# Autodesk Inventor assembly: mg996r leg top
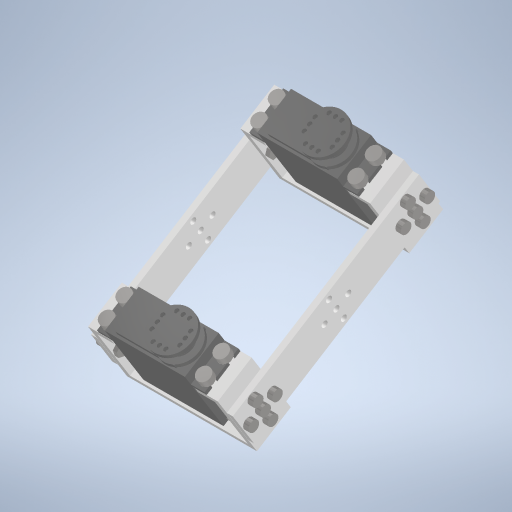
[picture p0: Inventor's stored thumbnail of the model, 512x512]
Saved by Autodesk Inventor 2023 (Build 270158000, 158)
## iProperties
Created: 2022-06-29
Part Number: mg996r leg top
Document SubType Name: Assembly
Designer: isamu
Author: isamu
## iProperties of the stored document Body008.ipt
Created: 2022-06-29
Part Number: Body008
Material: Generic
Document SubType Name: Modeling
Designer: isamu
Density: 1 g/cm^3
Appearance: Default
Author: isamu
## iProperties of the stored document servo frame part 4.iam
Created: 2022-07-03
Part Number: servo frame part 4
Description: FreeCAD Model
Document SubType Name: Assembly
Designer: isamu
Authority: Unknown
Sending System: FreeCAD
Preprocessor: Open CASCADE STEP processor 7.5
Title: Open CASCADE Shape Model
Author: Author
## Documents named in this file (7)
- **D:\personal_projects\robot\inventor\mg996r leg top.iam*LocalDocs*xAaaaafcaAaaaaaaaAaaaai2oXe*Body008.ipt
- **D:\personal_projects\robot\inventor\mg996r leg top.iam*LocalDocs*xAaaaajdaAaaaaaaaAaaaabubYc*servo frame part 4.iam
- D:\personal_projects\robot\inventor\mg996r leg top.iam
- D:\personal_projects\robot\exports\frames\m3x8.ipt
- D:\personal_projects\robot\exports\frames\m3 nuts.ipt
- D:\personal_projects\robot\inventor\base mg996r 3mm frame without axis.iam
- D:\personal_projects\robot\exports\frames\servo frame part 4.step
## Components (44 placed, 4 different names)
1. servo frame part 4:1 [sub-assembly] — Insert:26, Insert:27, Insert:28, Insert:29, Insert:30, Mate:1, Mate:7, Mate:8, Mate:9, Insert:41, Insert:42, Insert:43, Insert:44, Insert:45
2. servo frame part 4:2 [sub-assembly] — Insert:21, Insert:22, Insert:23, Insert:24, Insert:25, Mate:4, Insert:46, Insert:47, Insert:48, Insert:49, Insert:50
3. m3x8:1 — Insert:22, Mate:6
4. m3x8:2 — Insert:21, Mate:5
5. m3x8:3 — Insert:25
6. m3x8:4 — Insert:23
7. m3x8:5 — Insert:24
8. m3x8:6 — Insert:26, Mate:3
9. m3x8:7 — Insert:29
10. m3x8:8 — Insert:30
11. m3x8:9 — Insert:27, Mate:2
12. m3x8:10 — Insert:28
13. m3 nuts:1 — Insert:37
14. m3 nuts:2 — Insert:39
15. m3 nuts:3 — Insert:40
16. m3 nuts:4 — Insert:38
17. m3 nuts:5 — Insert:36
18. m3 nuts:6 — Insert:34
19. m3 nuts:7 — Insert:31
20. m3 nuts:8 — Insert:32
21. m3 nuts:9 — Insert:35
22. m3 nuts:10 — Insert:33
23. base mg996r 3mm frame without axis:1 [sub-assembly] — Mate:1, Mate:2, Mate:3, Mate:4, Mate:5, Mate:6, Insert:31, Insert:32, Insert:33, Insert:34, Insert:35, Insert:36, Insert:37, Insert:38, Insert:39, Insert:40
24. base mg996r 3mm frame without axis:2 [sub-assembly] — Mate:7, Mate:8, Mate:9, Insert:51, Insert:52, Insert:53, Insert:54, Insert:55, Insert:56, Insert:57, Insert:58, Insert:59, Insert:60
25. m3x8:11 — Insert:43
26. m3x8:12 — Insert:42
27. m3x8:13 — Insert:41
28. m3x8:14 — Insert:45
29. m3x8:15 — Insert:44
30. m3x8:16 — Insert:50
31. m3x8:17 — Insert:46
32. m3x8:18 — Insert:49
33. m3x8:19 — Insert:47
34. m3x8:20 — Insert:48
35. m3 nuts:11 — Insert:54
36. m3 nuts:12 — Insert:59
37. m3 nuts:13 — Insert:53
38. m3 nuts:14 — Insert:52
39. m3 nuts:15 — Insert:51
40. m3 nuts:16 — Insert:60
41. m3 nuts:17 — Insert:56
42. m3 nuts:18 — Insert:58
43. m3 nuts:19 — Insert:55
44. m3 nuts:20 — Insert:57
## Relationships (49: Insert 40, Mate 9)
- Insert:21: servo frame part 4:2 ↔ m3x8:2
- Insert:22: servo frame part 4:2 ↔ m3x8:1
- Insert:23: servo frame part 4:2 ↔ m3x8:4
- Insert:24: servo frame part 4:2 ↔ m3x8:5
- Insert:25: servo frame part 4:2 ↔ m3x8:3
- Insert:26: servo frame part 4:1 ↔ m3x8:6
- Insert:27: servo frame part 4:1 ↔ m3x8:9
- Insert:28: servo frame part 4:1 ↔ m3x8:10
- Insert:29: servo frame part 4:1 ↔ m3x8:7
- Insert:30: servo frame part 4:1 ↔ m3x8:8
- Mate:1: servo frame part 4:1 ↔ base mg996r 3mm frame without axis:1
- Mate:2: m3x8:9 ↔ base mg996r 3mm frame without axis:1
- Mate:3: m3x8:6 ↔ base mg996r 3mm frame without axis:1
- Mate:4: servo frame part 4:2 ↔ base mg996r 3mm frame without axis:1
- Mate:5: m3x8:2 ↔ base mg996r 3mm frame without axis:1
- Mate:6: m3x8:1 ↔ base mg996r 3mm frame without axis:1
- Insert:31: m3 nuts:7 ↔ base mg996r 3mm frame without axis:1
- Insert:32: m3 nuts:8 ↔ base mg996r 3mm frame without axis:1
- Insert:33: m3 nuts:10 ↔ base mg996r 3mm frame without axis:1
- Insert:34: m3 nuts:6 ↔ base mg996r 3mm frame without axis:1
- Insert:35: m3 nuts:9 ↔ base mg996r 3mm frame without axis:1
- Insert:36: m3 nuts:5 ↔ base mg996r 3mm frame without axis:1
- Insert:37: m3 nuts:1 ↔ base mg996r 3mm frame without axis:1
- Insert:38: m3 nuts:4 ↔ base mg996r 3mm frame without axis:1
- Insert:39: m3 nuts:2 ↔ base mg996r 3mm frame without axis:1
- Insert:40: m3 nuts:3 ↔ base mg996r 3mm frame without axis:1
- Mate:7: servo frame part 4:1 ↔ base mg996r 3mm frame without axis:2
- Mate:8: servo frame part 4:1 ↔ base mg996r 3mm frame without axis:2
- Mate:9: servo frame part 4:1 ↔ base mg996r 3mm frame without axis:2
- Insert:41: servo frame part 4:1 ↔ m3x8:13
- Insert:42: servo frame part 4:1 ↔ m3x8:12
- Insert:43: servo frame part 4:1 ↔ m3x8:11
- Insert:44: servo frame part 4:1 ↔ m3x8:15
- Insert:45: servo frame part 4:1 ↔ m3x8:14
- Insert:46: servo frame part 4:2 ↔ m3x8:17
- Insert:47: servo frame part 4:2 ↔ m3x8:19
- Insert:48: servo frame part 4:2 ↔ m3x8:20
- Insert:49: servo frame part 4:2 ↔ m3x8:18
- Insert:50: servo frame part 4:2 ↔ m3x8:16
- Insert:51: base mg996r 3mm frame without axis:2 ↔ m3 nuts:15
- Insert:52: base mg996r 3mm frame without axis:2 ↔ m3 nuts:14
- Insert:53: base mg996r 3mm frame without axis:2 ↔ m3 nuts:13
- Insert:54: base mg996r 3mm frame without axis:2 ↔ m3 nuts:11
- Insert:55: base mg996r 3mm frame without axis:2 ↔ m3 nuts:19
- Insert:56: base mg996r 3mm frame without axis:2 ↔ m3 nuts:17
- Insert:57: base mg996r 3mm frame without axis:2 ↔ m3 nuts:20
- Insert:58: base mg996r 3mm frame without axis:2 ↔ m3 nuts:18
- Insert:59: base mg996r 3mm frame without axis:2 ↔ m3 nuts:12
- Insert:60: base mg996r 3mm frame without axis:2 ↔ m3 nuts:16
